# Autodesk Inventor assembly: printer2
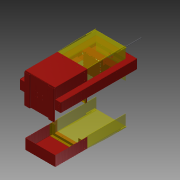
[picture p0: Inventor's stored thumbnail of the model, 180x180]
Saved by Autodesk Inventor 2014 SP2 (Build 180246200, 246)
## iProperties
Created: 2016-06-19
Part Number: printer2
Document SubType Name: Assembly
Designer: cruiser
Author: cruiser
## Documents named in this file (14)
- C:\Users\cruiser\Desktop\models\3d printers\laserresin4\printer2.iam
- C:\Users\cruiser\Desktop\models\3d printers\laserresin4\carrier2.ipt
- C:\Users\cruiser\Desktop\models\3d printers\laserresin4\frame_face2.ipt
- C:\Users\cruiser\Desktop\models\3d printers\laserresin4\door_assembly.iam
- C:\Users\cruiser\Desktop\models\3d printers\laserresin4\shf8.ipt
- C:\Users\cruiser\Desktop\models\3d printers\laserresin4\frame_back.ipt
- C:\Users\cruiser\Desktop\models\3d printers\laserresin4\crane_assembly.iam
- C:\Users\cruiser\Desktop\models\3d printers\laserresin4\reservoir.ipt
- C:\Users\cruiser\Desktop\models\3d printers\laserresin4\tray.ipt
- C:\Users\cruiser\Desktop\models\3d printers\laserresin4\laserholder.ipt
- C:\Users\cruiser\Desktop\models\3d printers\laserresin4\frame_feet.ipt
- C:\Users\cruiser\Desktop\models\3d printers\laserresin4\subframe.ipt
- C:\Users\cruiser\Desktop\models\3d printers\laserresin4\visor.ipt
- C:\Users\cruiser\Desktop\models\3d printers\laserresin4\threaded_rod.ipt
## Components (15 placed, 13 different names)
1. carrier2:1 — Mate:3, Mate:4, Mate:14, Mate:15, Mate:16, Mate:28, Mate:29, Mate:30, Mate:33, Mate:37
2. frame_face2:1 — Mate:1, Mate:2, Mate:5, Mate:6, Mate:7, Mate:8, Mate:9, Mate:10, Mate:11, Mate:12, Mate:13, Mate:20, Mate:21, Mate:22, Mate:23, Mate:24, Mate:25, Mate:26, Mate:28, Mate:29, Mate:30, Mate:34, Mate:35
3. door_assembly:1 [sub-assembly] — Mate:31, Mate:32, Mate:33
4. shf8:1 — Mate:1, Mate:2
5. frame_back:1 — Mate:20, Mate:21, Mate:22, Mate:23, Mate:24, Mate:27, Mate:32
6. crane_assembly:1 [sub-assembly] — Mate:34, Mate:35, Mate:38, Mate:39
7. reservoir:1 — Mate:14, Mate:15, Mate:16, Mate:17, Mate:18, Mate:19
8. tray:1 — Mate:17, Mate:18, Mate:19
9. shf8:2 — Mate:3, Mate:4
10. laserholder:1 — Mate:11, Mate:12, Mate:13
11. frame_feet:1 — Mate:5, Mate:6, Mate:7, Mate:31, Mate:36
12. subframe:1 — Mate:8, Mate:9, Mate:10
13. door_assembly:2 [sub-assembly] — Mate:36, Mate:37
14. visor:1 — Mate:25, Mate:26, Mate:27
15. threaded_rod:1 — Mate:38, Mate:39
## Relationships (39: Mate 39)
- Mate:1: frame_face2:1 ↔ shf8:1
- Mate:2: frame_face2:1 ↔ shf8:1
- Mate:3: carrier2:1 ↔ shf8:2
- Mate:4: carrier2:1 ↔ shf8:2
- Mate:5: frame_face2:1 ↔ frame_feet:1
- Mate:6: frame_face2:1 ↔ frame_feet:1
- Mate:7: frame_face2:1 ↔ frame_feet:1
- Mate:8: frame_face2:1 ↔ subframe:1
- Mate:9: frame_face2:1 ↔ subframe:1
- Mate:10: frame_face2:1 ↔ subframe:1
- Mate:11: frame_face2:1 ↔ laserholder:1
- Mate:12: frame_face2:1 ↔ laserholder:1
- Mate:13: frame_face2:1 ↔ laserholder:1
- Mate:14: carrier2:1 ↔ reservoir:1
- Mate:15: carrier2:1 ↔ reservoir:1
- Mate:16: carrier2:1 ↔ reservoir:1
- Mate:17: reservoir:1 ↔ tray:1
- Mate:18: reservoir:1 ↔ tray:1
- Mate:19: reservoir:1 ↔ tray:1
- Mate:20: frame_face2:1 ↔ frame_back:1
- Mate:21: frame_face2:1 ↔ frame_back:1
- Mate:22: frame_face2:1 ↔ frame_back:1
- Mate:23: frame_face2:1 ↔ frame_back:1
- Mate:24: frame_face2:1 ↔ frame_back:1
- Mate:25: frame_face2:1 ↔ visor:1
- Mate:26: frame_face2:1 ↔ visor:1
- Mate:27: frame_back:1 ↔ visor:1
- Mate:28: carrier2:1 ↔ frame_face2:1
- Mate:29: carrier2:1 ↔ frame_face2:1
- Mate:30: carrier2:1 ↔ frame_face2:1
- Mate:31: door_assembly:1 ↔ frame_feet:1
- Mate:32: door_assembly:1 ↔ frame_back:1
- Mate:33: carrier2:1 ↔ door_assembly:1
- Mate:34: frame_face2:1 ↔ crane_assembly:1
- Mate:35: frame_face2:1 ↔ crane_assembly:1
- Mate:36: frame_feet:1 ↔ door_assembly:2
- Mate:37: carrier2:1 ↔ door_assembly:2
- Mate:38: crane_assembly:1 ↔ threaded_rod:1
- Mate:39: crane_assembly:1 ↔ threaded_rod:1
